# Autodesk Inventor assembly: Pendolo_Inverso
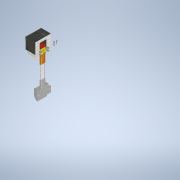
[picture p0: Inventor's stored thumbnail of the model, 180x180]
Saved by Autodesk Inventor 2020.2 (Build 242310000, 310)
## iProperties
Created: 2019-11-10
Part Number: Pendolo_Inverso
Document SubType Name: Assembly
Designer: socci
Author: socci
## Documents named in this file (20)
- C:\Users\socci\Desktop\mv-Project\04_PartDraw\Pendolo_Inverso.iam
- C:\Users\socci\Desktop\mv-Project\04_PartDraw\Componenti\19_Base_Pezzo_Unico.ipt
- C:\Users\socci\Documents\Inventor\Content Center Files\R2020\it-IT\Bearing GB_T 5800-2003\Rolling bearing GB_T 5800-2003 -635.ipt
- C:\Users\socci\Desktop\mv-Project\04_PartDraw\Componenti\1_Asse_cuscinetti.ipt
- C:\Users\socci\Desktop\mv-Project\04_PartDraw\Componenti\2_Connettore_inf_sup.ipt
- C:\Users\socci\Desktop\mv-Project\04_PartDraw\Componenti\3_Connettore_inf_INF.ipt
- C:\Users\socci\Desktop\mv-Project\04_PartDraw\Componenti\11_Connettore_MPU.ipt
- C:\Users\socci\Desktop\mv-Project\04_PartDraw\Componenti\10_MPU_6050.ipt
- C:\Users\socci\Desktop\mv-Project\04_PartDraw\Componenti\20_Base_Sopra.ipt
- C:\Users\socci\Desktop\mv-Project\04_PartDraw\Componenti\4_barra.ipt
- C:\Users\socci\Desktop\mv-Project\04_PartDraw\Componenti\22_Blocco_Escursione_Braccio.ipt
- C:\Users\socci\Desktop\mv-Project\04_PartDraw\Componenti\9_Flangia.ipt
- C:\Users\socci\Desktop\mv-Project\04_PartDraw\Componenti\24_Disco.ipt
- C:\Users\socci\Desktop\mv-Project\04_PartDraw\Componenti\26_Collana_di_Sfere.ipt
- C:\Users\socci\Documents\Inventor\Content Center Files\R2020\it-IT\DIN 1587\DIN 1587 - M6 x 1.ipt
- C:\Users\socci\Documents\Inventor\Content Center Files\R2020\it-IT\DIN 934\DIN 934 - M6 x 1.ipt
- C:\Users\socci\Desktop\mv-Project\04_PartDraw\Componenti\28_Rondella_M6.ipt
- C:\Users\socci\Documents\Inventor\Content Center Files\R2020\it-IT\DIN 933\DIN 933 - M6  x 30.ipt
- C:\Users\socci\Desktop\mv-Project\04_PartDraw\Componenti\30_Connettore_sup.ipt
- C:\Users\socci\Desktop\mv-Project\04_PartDraw\Componenti\29_Motore_6mm.ipt
## Components (163 placed, 19 different names)
1. 19_Base_Pezzo_Unico:1 — Inserimento:1, Inserimento:2, Angolo:1, Coincidente:3, Coincidente:4, Coincidente:11, Coincidente:12, Allineato:4, Allineato:14, Coincidente:14, Coincidente:15, Allineato:5
2. Bearing GB/T 5800-2003 635:1 — Inserimento:1, Inserimento:3, Inserimento:9
3. Bearing GB/T 5800-2003 635:2 — Inserimento:2, Inserimento:4, Inserimento:8
4. 1_Asse_cuscinetti:1 — Inserimento:3, Inserimento:4, Inserimento:5, Inserimento:6, Inserimento:7
5. 2_Connettore_inf_sup:1 — Inserimento:6, Coincidente:1, Angolo:1, Allineato:3, Coincidente:5, Coincidente:6, Coincidente:7
6. 3_Connettore_inf_INF:1 — Inserimento:5, Coincidente:1
7. 11_Connettore_MPU:1 — Coincidente:2, Allineato:1, Allineato:2, Allineato:3, Inserimento:7
8. 10_MPU_6050:1 — Coincidente:2, Allineato:1, Allineato:2
9. 20_Base_Sopra:1 — Coincidente:3, Inserimento:9
10. 20_Base_Sopra:2 — Coincidente:4, Inserimento:8
11. 4_barra:1 — Coincidente:5, Coincidente:6, Coincidente:7, Coincidente:19, Coincidente:20, Coincidente:21
12. 22_Blocco_Escursione_Braccio:1 — Coincidente:11, Coincidente:12, Allineato:4
13. 22_Blocco_Escursione_Braccio:2 — Coincidente:14, Coincidente:15, Allineato:5
14. 9_Flangia:1
15. 30_Connettore_sup:1 — Coincidente:19, Coincidente:20, Coincidente:21, Inserimento:318
16. 29_Motore_6mm:1 — Inserimento:318
17. 24_Disco:1
18. 24_Disco:2 — Inserimento:316, Inserimento:317
19. DIN 1587 M6:1
20. DIN 934 - sostituito da DIN EN 24032/28673/28674 M6:1
21. 28_Rondella_M6:1
22. DIN 933 - sostituito da DIN EN 24017 M6  x 30:1
23. 28_Rondella_M6:2
24. 28_Rondella_M6:3
25. 28_Rondella_M6:4
26. 28_Rondella_M6:5
27. 28_Rondella_M6:6
28. DIN 1587 M6:2
29. DIN 934 - sostituito da DIN EN 24032/28673/28674 M6:2
30. 28_Rondella_M6:7
31. DIN 933 - sostituito da DIN EN 24017 M6  x 30:2
32. 28_Rondella_M6:8
33. 28_Rondella_M6:9
34. 28_Rondella_M6:10
35. 28_Rondella_M6:11
36. 28_Rondella_M6:12
37. DIN 1587 M6:3
38. DIN 934 - sostituito da DIN EN 24032/28673/28674 M6:3
39. 28_Rondella_M6:13
40. DIN 933 - sostituito da DIN EN 24017 M6  x 30:3
41. 28_Rondella_M6:14
42. 28_Rondella_M6:15
43. 28_Rondella_M6:16
44. 28_Rondella_M6:17
45. 28_Rondella_M6:18
46. DIN 1587 M6:4
47. DIN 934 - sostituito da DIN EN 24032/28673/28674 M6:4
48. 28_Rondella_M6:19
49. DIN 933 - sostituito da DIN EN 24017 M6  x 30:4
50. 28_Rondella_M6:20
51. 28_Rondella_M6:21
52. 28_Rondella_M6:22
53. 28_Rondella_M6:23
54. 28_Rondella_M6:24
55. DIN 1587 M6:5
56. DIN 934 - sostituito da DIN EN 24032/28673/28674 M6:5
57. 28_Rondella_M6:25
58. DIN 933 - sostituito da DIN EN 24017 M6  x 30:5
59. 28_Rondella_M6:26
60. 28_Rondella_M6:27
61. 28_Rondella_M6:28
62. 28_Rondella_M6:29
63. 28_Rondella_M6:30
64. DIN 1587 M6:6
65. DIN 934 - sostituito da DIN EN 24032/28673/28674 M6:6
66. 28_Rondella_M6:31
67. DIN 933 - sostituito da DIN EN 24017 M6  x 30:6
68. 28_Rondella_M6:32
69. 28_Rondella_M6:33
70. 28_Rondella_M6:34
71. 28_Rondella_M6:35
72. 28_Rondella_M6:36
73. DIN 1587 M6:7
74. DIN 934 - sostituito da DIN EN 24032/28673/28674 M6:7
75. 28_Rondella_M6:37
76. DIN 933 - sostituito da DIN EN 24017 M6  x 30:7
77. 28_Rondella_M6:38
78. 28_Rondella_M6:39
79. 28_Rondella_M6:40
80. 28_Rondella_M6:41
81. 28_Rondella_M6:42
82. DIN 1587 M6:8
83. DIN 934 - sostituito da DIN EN 24032/28673/28674 M6:8
84. 28_Rondella_M6:43
85. DIN 933 - sostituito da DIN EN 24017 M6  x 30:8
86. 28_Rondella_M6:44
87. 28_Rondella_M6:45
88. 28_Rondella_M6:46
89. 28_Rondella_M6:47
90. 28_Rondella_M6:48
91. DIN 1587 M6:9
92. DIN 934 - sostituito da DIN EN 24032/28673/28674 M6:9
93. 28_Rondella_M6:49
94. DIN 933 - sostituito da DIN EN 24017 M6  x 30:9
95. 28_Rondella_M6:50
96. 28_Rondella_M6:51
97. 28_Rondella_M6:52
98. 28_Rondella_M6:53
99. 28_Rondella_M6:54
100. DIN 1587 M6:10
101. DIN 934 - sostituito da DIN EN 24032/28673/28674 M6:10
102. 28_Rondella_M6:55
103. DIN 933 - sostituito da DIN EN 24017 M6  x 30:10
104. 28_Rondella_M6:56
105. 28_Rondella_M6:57
106. 28_Rondella_M6:58
107. 28_Rondella_M6:59
108. 28_Rondella_M6:60
109. DIN 1587 M6:11
110. DIN 934 - sostituito da DIN EN 24032/28673/28674 M6:11
111. 28_Rondella_M6:61
112. DIN 933 - sostituito da DIN EN 24017 M6  x 30:11
113. 28_Rondella_M6:62
114. 28_Rondella_M6:63
115. 28_Rondella_M6:64
116. 28_Rondella_M6:65
117. 28_Rondella_M6:66
118. DIN 1587 M6:12
119. DIN 934 - sostituito da DIN EN 24032/28673/28674 M6:12
120. 28_Rondella_M6:67
121. DIN 933 - sostituito da DIN EN 24017 M6  x 30:12
122. 28_Rondella_M6:68
123. 28_Rondella_M6:69
124. 28_Rondella_M6:70
125. 28_Rondella_M6:71
126. 28_Rondella_M6:72
127. DIN 1587 M6:13
128. DIN 934 - sostituito da DIN EN 24032/28673/28674 M6:13
129. 28_Rondella_M6:73
130. DIN 933 - sostituito da DIN EN 24017 M6  x 30:13
131. 28_Rondella_M6:74
132. 28_Rondella_M6:75
133. 28_Rondella_M6:76
134. 28_Rondella_M6:77
135. 28_Rondella_M6:78
136. DIN 1587 M6:14
137. DIN 934 - sostituito da DIN EN 24032/28673/28674 M6:14
138. 28_Rondella_M6:79
139. DIN 933 - sostituito da DIN EN 24017 M6  x 30:14
140. 28_Rondella_M6:80
141. 28_Rondella_M6:81
142. 28_Rondella_M6:82
143. 28_Rondella_M6:83
144. 28_Rondella_M6:84
145. DIN 1587 M6:15
146. DIN 934 - sostituito da DIN EN 24032/28673/28674 M6:15
147. 28_Rondella_M6:85
148. DIN 933 - sostituito da DIN EN 24017 M6  x 30:15
149. 28_Rondella_M6:86
150. 28_Rondella_M6:87
151. 28_Rondella_M6:88
152. 28_Rondella_M6:89
153. 28_Rondella_M6:90
154. DIN 1587 M6:16
155. DIN 934 - sostituito da DIN EN 24032/28673/28674 M6:16
156. 28_Rondella_M6:91
157. DIN 933 - sostituito da DIN EN 24017 M6  x 30:16
158. 28_Rondella_M6:92
159. 28_Rondella_M6:93
160. 28_Rondella_M6:94
161. 28_Rondella_M6:95
162. 28_Rondella_M6:96
163. 26_Collana_di_Sfere:1 — Inserimento:316, Inserimento:317
## Relationships (184: Insert 162, Mate 15, Flush 6, Angle 1)
- Inserimento:1: 19_Base_Pezzo_Unico:1 ↔ Bearing GB/T 5800-2003 635:1
- Inserimento:2: 19_Base_Pezzo_Unico:1 ↔ Bearing GB/T 5800-2003 635:2
- Inserimento:3 (1.5 mm): Bearing GB/T 5800-2003 635:1 ↔ 1_Asse_cuscinetti:1
- Inserimento:4 (2.5 mm): Bearing GB/T 5800-2003 635:2 ↔ 1_Asse_cuscinetti:1
- Inserimento:5: 1_Asse_cuscinetti:1 ↔ 3_Connettore_inf_INF:1
- Inserimento:6: 1_Asse_cuscinetti:1 ↔ 2_Connettore_inf_sup:1
- Coincidente:1 [Mate] (1 mm): 2_Connettore_inf_sup:1 ↔ 3_Connettore_inf_INF:1
- Coincidente:2 [Mate] (10 mm): 11_Connettore_MPU:1 ↔ 10_MPU_6050:1
- Allineato:1 [Flush] (2 mm): 11_Connettore_MPU:1 ↔ 10_MPU_6050:1
- Allineato:2 [Flush] (3 mm): 11_Connettore_MPU:1 ↔ 10_MPU_6050:1
- Angolo:1 [Angle] (0 deg): 19_Base_Pezzo_Unico:1 ↔ 2_Connettore_inf_sup:1
- Allineato:3 [Flush] (-9.5 mm): 2_Connettore_inf_sup:1 ↔ 11_Connettore_MPU:1
- Inserimento:7: 1_Asse_cuscinetti:1 ↔ 11_Connettore_MPU:1
- Coincidente:3 [Mate] (1 mm): 19_Base_Pezzo_Unico:1 ↔ 20_Base_Sopra:1
- Coincidente:4 [Mate] (1 mm): 19_Base_Pezzo_Unico:1 ↔ 20_Base_Sopra:2
- Inserimento:8: Bearing GB/T 5800-2003 635:2 ↔ 20_Base_Sopra:2
- Inserimento:9: Bearing GB/T 5800-2003 635:1 ↔ 20_Base_Sopra:1
- Coincidente:5 [Mate] (0.5 mm): 2_Connettore_inf_sup:1 ↔ 4_barra:1
- Coincidente:6 [Mate] (0.5 mm): 2_Connettore_inf_sup:1 ↔ 4_barra:1
- Coincidente:7 [Mate]: 2_Connettore_inf_sup:1 ↔ 4_barra:1
- Coincidente:11 [Mate]: 19_Base_Pezzo_Unico:1 ↔ 22_Blocco_Escursione_Braccio:1
- Coincidente:12 [Mate] (0.2 mm): 19_Base_Pezzo_Unico:1 ↔ 22_Blocco_Escursione_Braccio:1
- Allineato:4 [Flush]: 19_Base_Pezzo_Unico:1 ↔ 22_Blocco_Escursione_Braccio:1
- Allineato:14 [Flush]: 19_Base_Pezzo_Unico:1
- Coincidente:14 [Mate] (0.2 mm): 19_Base_Pezzo_Unico:1 ↔ 22_Blocco_Escursione_Braccio:2
- Coincidente:15 [Mate]: 19_Base_Pezzo_Unico:1 ↔ 22_Blocco_Escursione_Braccio:2
- Allineato:5 [Flush]: 19_Base_Pezzo_Unico:1 ↔ 22_Blocco_Escursione_Braccio:2
- [Insert] (7.829 mm): 24_Disco:1 ↔ 24_Disco:2
- [Insert] (7.829 mm): 24_Disco:1 ↔ 24_Disco:2
- [Insert] (7.829 mm): 24_Disco:1 ↔ 24_Disco:2
- [Insert] (7.829 mm): 24_Disco:1 ↔ 24_Disco:2
- [Insert]: 28_Rondella_M6:1 ↔ DIN 933 - sostituito da DIN EN 24017 M6  x 30:1
- [Insert] (4 mm): 28_Rondella_M6:1 ↔ 28_Rondella_M6:2
- [Insert]: DIN 934 - sostituito da DIN EN 24032/28673/28674 M6:1 ↔ 28_Rondella_M6:2
- [Insert]: DIN 934 - sostituito da DIN EN 24032/28673/28674 M6:1 ↔ 28_Rondella_M6:3
- [Insert] (4 mm): 28_Rondella_M6:3 ↔ 28_Rondella_M6:5
- [Insert]: 28_Rondella_M6:5 ↔ 28_Rondella_M6:6
- [Insert]: 28_Rondella_M6:4 ↔ 28_Rondella_M6:6
- [Insert]: DIN 1587 M6:1 ↔ 28_Rondella_M6:4
- [Insert]: 28_Rondella_M6:7 ↔ DIN 933 - sostituito da DIN EN 24017 M6  x 30:2
- [Insert] (4 mm): 28_Rondella_M6:7 ↔ 28_Rondella_M6:8
- [Insert]: DIN 934 - sostituito da DIN EN 24032/28673/28674 M6:2 ↔ 28_Rondella_M6:8
- [Insert]: DIN 934 - sostituito da DIN EN 24032/28673/28674 M6:2 ↔ 28_Rondella_M6:9
- [Insert] (4 mm): 28_Rondella_M6:9 ↔ 28_Rondella_M6:11
- [Insert]: 28_Rondella_M6:11 ↔ 28_Rondella_M6:12
- [Insert]: 28_Rondella_M6:10 ↔ 28_Rondella_M6:12
- [Insert]: DIN 1587 M6:2 ↔ 28_Rondella_M6:10
- [Insert]: 24_Disco:2 ↔ 28_Rondella_M6:7
- [Insert]: 28_Rondella_M6:13 ↔ DIN 933 - sostituito da DIN EN 24017 M6  x 30:3
- [Insert] (4 mm): 28_Rondella_M6:13 ↔ 28_Rondella_M6:14
- [Insert]: DIN 934 - sostituito da DIN EN 24032/28673/28674 M6:3 ↔ 28_Rondella_M6:14
- [Insert]: DIN 934 - sostituito da DIN EN 24032/28673/28674 M6:3 ↔ 28_Rondella_M6:15
- [Insert] (4 mm): 28_Rondella_M6:15 ↔ 28_Rondella_M6:17
- [Insert]: 28_Rondella_M6:17 ↔ 28_Rondella_M6:18
- [Insert]: 28_Rondella_M6:16 ↔ 28_Rondella_M6:18
- [Insert]: DIN 1587 M6:3 ↔ 28_Rondella_M6:16
- [Insert]: 28_Rondella_M6:19 ↔ DIN 933 - sostituito da DIN EN 24017 M6  x 30:4
- [Insert] (4 mm): 28_Rondella_M6:19 ↔ 28_Rondella_M6:20
- [Insert]: DIN 934 - sostituito da DIN EN 24032/28673/28674 M6:4 ↔ 28_Rondella_M6:20
- [Insert]: DIN 934 - sostituito da DIN EN 24032/28673/28674 M6:4 ↔ 28_Rondella_M6:21
- [Insert] (4 mm): 28_Rondella_M6:21 ↔ 28_Rondella_M6:23
- [Insert]: 28_Rondella_M6:23 ↔ 28_Rondella_M6:24
- [Insert]: 28_Rondella_M6:22 ↔ 28_Rondella_M6:24
- [Insert]: DIN 1587 M6:4 ↔ 28_Rondella_M6:22
- [Insert]: 28_Rondella_M6:25 ↔ DIN 933 - sostituito da DIN EN 24017 M6  x 30:5
- [Insert] (4 mm): 28_Rondella_M6:25 ↔ 28_Rondella_M6:26
- [Insert]: DIN 934 - sostituito da DIN EN 24032/28673/28674 M6:5 ↔ 28_Rondella_M6:26
- [Insert]: DIN 934 - sostituito da DIN EN 24032/28673/28674 M6:5 ↔ 28_Rondella_M6:27
- [Insert] (4 mm): 28_Rondella_M6:27 ↔ 28_Rondella_M6:29
- [Insert]: 28_Rondella_M6:29 ↔ 28_Rondella_M6:30
- [Insert]: 28_Rondella_M6:28 ↔ 28_Rondella_M6:30
- [Insert]: DIN 1587 M6:5 ↔ 28_Rondella_M6:28
- [Insert]: 28_Rondella_M6:31 ↔ DIN 933 - sostituito da DIN EN 24017 M6  x 30:6
- [Insert] (4 mm): 28_Rondella_M6:31 ↔ 28_Rondella_M6:32
- [Insert]: DIN 934 - sostituito da DIN EN 24032/28673/28674 M6:6 ↔ 28_Rondella_M6:32
- [Insert]: DIN 934 - sostituito da DIN EN 24032/28673/28674 M6:6 ↔ 28_Rondella_M6:33
- [Insert] (4 mm): 28_Rondella_M6:33 ↔ 28_Rondella_M6:35
- [Insert]: 28_Rondella_M6:35 ↔ 28_Rondella_M6:36
- [Insert]: 28_Rondella_M6:34 ↔ 28_Rondella_M6:36
- [Insert]: DIN 1587 M6:6 ↔ 28_Rondella_M6:34
- [Insert]: 28_Rondella_M6:37 ↔ DIN 933 - sostituito da DIN EN 24017 M6  x 30:7
- [Insert] (4 mm): 28_Rondella_M6:37 ↔ 28_Rondella_M6:38
- [Insert]: DIN 934 - sostituito da DIN EN 24032/28673/28674 M6:7 ↔ 28_Rondella_M6:38
- [Insert]: DIN 934 - sostituito da DIN EN 24032/28673/28674 M6:7 ↔ 28_Rondella_M6:39
- [Insert] (4 mm): 28_Rondella_M6:39 ↔ 28_Rondella_M6:41
- [Insert]: 28_Rondella_M6:41 ↔ 28_Rondella_M6:42
- [Insert]: 28_Rondella_M6:40 ↔ 28_Rondella_M6:42
- [Insert]: DIN 1587 M6:7 ↔ 28_Rondella_M6:40
- [Insert]: 28_Rondella_M6:43 ↔ DIN 933 - sostituito da DIN EN 24017 M6  x 30:8
- [Insert] (4 mm): 28_Rondella_M6:43 ↔ 28_Rondella_M6:44
- [Insert]: DIN 934 - sostituito da DIN EN 24032/28673/28674 M6:8 ↔ 28_Rondella_M6:44
- [Insert]: DIN 934 - sostituito da DIN EN 24032/28673/28674 M6:8 ↔ 28_Rondella_M6:45
- [Insert] (4 mm): 28_Rondella_M6:45 ↔ 28_Rondella_M6:47
- [Insert]: 28_Rondella_M6:47 ↔ 28_Rondella_M6:48
- [Insert]: 28_Rondella_M6:46 ↔ 28_Rondella_M6:48
- [Insert]: DIN 1587 M6:8 ↔ 28_Rondella_M6:46
- [Insert]: 28_Rondella_M6:49 ↔ DIN 933 - sostituito da DIN EN 24017 M6  x 30:9
- [Insert] (4 mm): 28_Rondella_M6:49 ↔ 28_Rondella_M6:50
- [Insert]: DIN 934 - sostituito da DIN EN 24032/28673/28674 M6:9 ↔ 28_Rondella_M6:50
- [Insert]: DIN 934 - sostituito da DIN EN 24032/28673/28674 M6:9 ↔ 28_Rondella_M6:51
- [Insert] (4 mm): 28_Rondella_M6:51 ↔ 28_Rondella_M6:53
- [Insert]: 28_Rondella_M6:53 ↔ 28_Rondella_M6:54
- [Insert]: 28_Rondella_M6:52 ↔ 28_Rondella_M6:54
- [Insert]: DIN 1587 M6:9 ↔ 28_Rondella_M6:52
- [Insert]: 28_Rondella_M6:55 ↔ DIN 933 - sostituito da DIN EN 24017 M6  x 30:10
- [Insert] (4 mm): 28_Rondella_M6:55 ↔ 28_Rondella_M6:56
- [Insert]: DIN 934 - sostituito da DIN EN 24032/28673/28674 M6:10 ↔ 28_Rondella_M6:56
- [Insert]: DIN 934 - sostituito da DIN EN 24032/28673/28674 M6:10 ↔ 28_Rondella_M6:57
- [Insert] (4 mm): 28_Rondella_M6:57 ↔ 28_Rondella_M6:59
- [Insert]: 28_Rondella_M6:59 ↔ 28_Rondella_M6:60
- [Insert]: 28_Rondella_M6:58 ↔ 28_Rondella_M6:60
- [Insert]: DIN 1587 M6:10 ↔ 28_Rondella_M6:58
- [Insert]: 28_Rondella_M6:61 ↔ DIN 933 - sostituito da DIN EN 24017 M6  x 30:11
- [Insert] (4 mm): 28_Rondella_M6:61 ↔ 28_Rondella_M6:62
- [Insert]: DIN 934 - sostituito da DIN EN 24032/28673/28674 M6:11 ↔ 28_Rondella_M6:62
- [Insert]: DIN 934 - sostituito da DIN EN 24032/28673/28674 M6:11 ↔ 28_Rondella_M6:63
- [Insert] (4 mm): 28_Rondella_M6:63 ↔ 28_Rondella_M6:65
- [Insert]: 28_Rondella_M6:65 ↔ 28_Rondella_M6:66
- [Insert]: 28_Rondella_M6:64 ↔ 28_Rondella_M6:66
- [Insert]: DIN 1587 M6:11 ↔ 28_Rondella_M6:64
- [Insert]: 28_Rondella_M6:67 ↔ DIN 933 - sostituito da DIN EN 24017 M6  x 30:12
- [Insert] (4 mm): 28_Rondella_M6:67 ↔ 28_Rondella_M6:68
- [Insert]: DIN 934 - sostituito da DIN EN 24032/28673/28674 M6:12 ↔ 28_Rondella_M6:68
- [Insert]: DIN 934 - sostituito da DIN EN 24032/28673/28674 M6:12 ↔ 28_Rondella_M6:69
- [Insert] (4 mm): 28_Rondella_M6:69 ↔ 28_Rondella_M6:71
- [Insert]: 28_Rondella_M6:71 ↔ 28_Rondella_M6:72
- [Insert]: 28_Rondella_M6:70 ↔ 28_Rondella_M6:72
- [Insert]: DIN 1587 M6:12 ↔ 28_Rondella_M6:70
- [Insert]: 28_Rondella_M6:73 ↔ DIN 933 - sostituito da DIN EN 24017 M6  x 30:13
- [Insert] (4 mm): 28_Rondella_M6:73 ↔ 28_Rondella_M6:74
- [Insert]: DIN 934 - sostituito da DIN EN 24032/28673/28674 M6:13 ↔ 28_Rondella_M6:74
- [Insert]: DIN 934 - sostituito da DIN EN 24032/28673/28674 M6:13 ↔ 28_Rondella_M6:75
- [Insert] (4 mm): 28_Rondella_M6:75 ↔ 28_Rondella_M6:77
- [Insert]: 28_Rondella_M6:77 ↔ 28_Rondella_M6:78
- [Insert]: 28_Rondella_M6:76 ↔ 28_Rondella_M6:78
- [Insert]: DIN 1587 M6:13 ↔ 28_Rondella_M6:76
- [Insert]: 28_Rondella_M6:79 ↔ DIN 933 - sostituito da DIN EN 24017 M6  x 30:14
- [Insert] (4 mm): 28_Rondella_M6:79 ↔ 28_Rondella_M6:80
- [Insert]: DIN 934 - sostituito da DIN EN 24032/28673/28674 M6:14 ↔ 28_Rondella_M6:80
- [Insert]: DIN 934 - sostituito da DIN EN 24032/28673/28674 M6:14 ↔ 28_Rondella_M6:81
- [Insert] (4 mm): 28_Rondella_M6:81 ↔ 28_Rondella_M6:83
- [Insert]: 28_Rondella_M6:83 ↔ 28_Rondella_M6:84
- [Insert]: 28_Rondella_M6:82 ↔ 28_Rondella_M6:84
- [Insert]: DIN 1587 M6:14 ↔ 28_Rondella_M6:82
- [Insert]: 28_Rondella_M6:85 ↔ DIN 933 - sostituito da DIN EN 24017 M6  x 30:15
- [Insert] (4 mm): 28_Rondella_M6:85 ↔ 28_Rondella_M6:86
- [Insert]: DIN 934 - sostituito da DIN EN 24032/28673/28674 M6:15 ↔ 28_Rondella_M6:86
- [Insert]: DIN 934 - sostituito da DIN EN 24032/28673/28674 M6:15 ↔ 28_Rondella_M6:87
- [Insert] (4 mm): 28_Rondella_M6:87 ↔ 28_Rondella_M6:89
- [Insert]: 28_Rondella_M6:89 ↔ 28_Rondella_M6:90
- [Insert]: 28_Rondella_M6:88 ↔ 28_Rondella_M6:90
- [Insert]: DIN 1587 M6:15 ↔ 28_Rondella_M6:88
- [Insert]: 28_Rondella_M6:91 ↔ DIN 933 - sostituito da DIN EN 24017 M6  x 30:16
- [Insert] (4 mm): 28_Rondella_M6:91 ↔ 28_Rondella_M6:92
- [Insert]: DIN 934 - sostituito da DIN EN 24032/28673/28674 M6:16 ↔ 28_Rondella_M6:92
- [Insert]: DIN 934 - sostituito da DIN EN 24032/28673/28674 M6:16 ↔ 28_Rondella_M6:93
- [Insert] (4 mm): 28_Rondella_M6:93 ↔ 28_Rondella_M6:95
- [Insert]: 28_Rondella_M6:95 ↔ 28_Rondella_M6:96
- [Insert]: 28_Rondella_M6:94 ↔ 28_Rondella_M6:96
- [Insert]: DIN 1587 M6:16 ↔ 28_Rondella_M6:94
- [Insert]: 24_Disco:2 ↔ 28_Rondella_M6:1
- [Insert]: 24_Disco:2 ↔ 28_Rondella_M6:91
- [Insert]: 24_Disco:2 ↔ 28_Rondella_M6:19
- [Insert]: 24_Disco:2 ↔ 28_Rondella_M6:43
- [Insert]: 24_Disco:2 ↔ 28_Rondella_M6:49
- [Insert]: 24_Disco:2 ↔ 28_Rondella_M6:55
- [Insert]: 24_Disco:2 ↔ 28_Rondella_M6:67
- [Insert]: 24_Disco:2 ↔ 28_Rondella_M6:79
- [Insert]: 24_Disco:2 ↔ 28_Rondella_M6:85
- [Insert]: 24_Disco:2 ↔ 28_Rondella_M6:73
- [Insert]: 24_Disco:2 ↔ 28_Rondella_M6:37
- [Insert]: 24_Disco:2 ↔ 28_Rondella_M6:61
- [Insert]: 24_Disco:2 ↔ 28_Rondella_M6:25
- [Insert]: 24_Disco:2 ↔ 28_Rondella_M6:13
- [Insert]: 24_Disco:2 ↔ 28_Rondella_M6:31
- [Mate]: 9_Flangia:1 ↔ 24_Disco:2
- [Insert]: 9_Flangia:1 ↔ 24_Disco:2
- [Insert]: 9_Flangia:1 ↔ 24_Disco:2
- Inserimento:316: 24_Disco:2 ↔ 26_Collana_di_Sfere:1
- Inserimento:317: 24_Disco:2 ↔ 26_Collana_di_Sfere:1
- Coincidente:19 [Mate]: 4_barra:1 ↔ 30_Connettore_sup:1
- Coincidente:20 [Mate]: 4_barra:1 ↔ 30_Connettore_sup:1
- Coincidente:21 [Mate]: 4_barra:1 ↔ 30_Connettore_sup:1
- Inserimento:318: 30_Connettore_sup:1 ↔ 29_Motore_6mm:1
## Named parameters: d362_d2 = 7.829 mm, d363_d3 = 7.829 mm, d103_d6 = 0 mm, d104_d7 = 4 mm, d105_d8 = 0 mm, d106_d9 = 0 mm, d107_d10 = 4 mm, d108_d11 = 0 mm, d109_d12 = 0 mm, d110_d13 = 0 mm, d111_d6 = 0 mm, d112_d7 = 4 mm, d113_d8 = 0 mm, d114_d9 = 0 mm, d115_d10 = 4 mm, d116_d11 = 0 mm, d117_d12 = 0 mm, d118_d13 = 0 mm, d119_d6 = 0 mm, d120_d7 = 4 mm, d121_d8 = 0 mm, d122_d9 = 0 mm, d123_d10 = 4 mm, d124_d11 = 0 mm, d125_d12 = 0 mm, d126_d13 = 0 mm, d127_d6 = 0 mm, d128_d7 = 4 mm, d129_d8 = 0 mm, d130_d9 = 0 mm, d131_d10 = 4 mm, d132_d11 = 0 mm, d133_d12 = 0 mm, d134_d13 = 0 mm, d65_d8 = 0 mm, d66_d9 = 0 mm, d67_d10 = 4 mm, d68_d11 = 0 mm, d69_d12 = 0 mm, d70_d13 = 0 mm, d71_d6 = 0 mm, d72_d7 = 4 mm, d73_d8 = 0 mm, d74_d9 = 0 mm, d75_d10 = 4 mm, d76_d11 = 0 mm, d77_d12 = 0 mm, d78_d13 = 0 mm, d79_d6 = 0 mm, d80_d7 = 4 mm, d81_d8 = 0 mm, d82_d9 = 0 mm, d83_d10 = 4 mm, d84_d11 = 0 mm, d85_d12 = 0 mm, d86_d13 = 0 mm, d87_d6 = 0 mm, d88_d7 = 4 mm, d89_d8 = 0 mm, d90_d9 = 0 mm, d91_d10 = 4 mm, d92_d11 = 0 mm, d93_d12 = 0 mm, d94_d13 = 0 mm, d95_d6 = 0 mm, d96_d7 = 4 mm, d97_d8 = 0 mm, d98_d9 = 0 mm, d99_d10 = 4 mm, d100_d11 = 0 mm, d101_d12 = 0 mm, d102_d13 = 0 mm, d31_d6 = 0 mm, d32_d7 = 4 mm, d33_d8 = 0 mm, d34_d9 = 0 mm, d35_d10 = 4 mm, d36_d11 = 0 mm, d37_d12 = 0 mm, d38_d13 = 0 mm, d39_d6 = 0 mm, d40_d7 = 4 mm, d41_d8 = 0 mm, d42_d9 = 0 mm, d43_d10 = 4 mm, d44_d11 = 0 mm, d45_d12 = 0 mm, d46_d13 = 0 mm, d47_d6 = 0 mm, d48_d7 = 4 mm, d49_d8 = 0 mm, d50_d9 = 0 mm, d51_d10 = 4 mm, d52_d11 = 0 mm, d53_d12 = 0 mm, d54_d13 = 0 mm, d55_d6 = 0 mm, d56_d7 = 4 mm, d57_d8 = 0 mm, d58_d9 = 0 mm, d59_d10 = 4 mm, d60_d11 = 0 mm, d61_d12 = 0 mm, d62_d13 = 0 mm, d63_d6 = 0 mm, d64_d7 = 4 mm, d485_d6 = 0 mm, d486_d7 = 4 mm, d487_d8 = 0 mm, d489_d10 = 4 mm, d490_d11 = 0 mm, d491_d12 = 0 mm, d492_d13 = 0 mm, d14_d6 = 0 mm, d15_d7 = 4 mm, d16_d8 = 0 mm, d17_d9 = 0 mm, d18_d10 = 4 mm, d19_d11 = 0 mm, d20_d12 = 0 mm, d21_d13 = 0 mm, d501_d22 = 0 mm, d23_d6 = 0 mm, d24_d7 = 4 mm, d25_d8 = 0 mm, d26_d9 = 0 mm, d27_d10 = 4 mm, d28_d11 = 0 mm, d29_d12 = 0 mm, d30_d13 = 0 mm
